# Autodesk Inventor assembly: Assembly_USB_Lampassembly
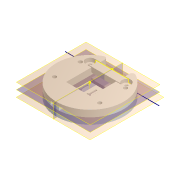
[picture p0: Inventor's stored thumbnail of the model, 180x180]
Saved by Autodesk Inventor 2022 (Build 260153000, 153)
## iProperties
Created: 2022-12-21
Part Number: Assembly_USB_Lampassembly
Document SubType Name: Assembly
Designer: diederichbenedict
Author: diederichbenedict
## Documents named in this file (4)
- C:\Users\diederichbenedict\Dropbox\Dokumente\Promotion\PROJECTS\Matchboxscope\INVENTOR\MATCHBOXSCOPE\Assembly_USB_Lampassembly.iam
- C:\Users\diederichbenedict\Dropbox\Dokumente\Promotion\PROJECTS\Matchboxscope\INVENTOR\MATCHBOXSCOPE\Matchboxscope_layer_ikealamp.ipt
- C:\Users\diederichbenedict\Dropbox\Dokumente\Promotion\PROJECTS\Matchboxscope\INVENTOR\Planktoscope_Mini\USB_dupont_Adapter.ipt
- C:\Users\diederichbenedict\Dropbox\Dokumente\Promotion\PROJECTS\Matchboxscope\INVENTOR\MATCHBOXSCOPE\Cableholder_Ikealamp.ipt
## Components (3 placed, 3 different names)
1. Matchboxscope_layer_ikealamp:1 — Passend:1, Fluchtend:2, Fluchtend:3
2. USB_dupont_Adapter:1 — Passend:1, Fluchtend:1
3. Cableholder_Ikealamp:1 — Fluchtend:2, Fluchtend:3
## Relationships (4: Flush 3, Mate 1)
- Passend:1 [Mate]: Matchboxscope_layer_ikealamp:1 ↔ USB_dupont_Adapter:1
- Fluchtend:1 [Flush] (-5 mm): USB_dupont_Adapter:1
- Fluchtend:2 [Flush]: Matchboxscope_layer_ikealamp:1 ↔ Cableholder_Ikealamp:1
- Fluchtend:3 [Flush]: Matchboxscope_layer_ikealamp:1 ↔ Cableholder_Ikealamp:1
